# Autodesk Inventor assembly: Wheel Assembly
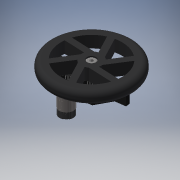
[picture p0: Inventor's stored thumbnail of the model, 180x180]
Saved by Autodesk Inventor 2017 (Build 210142000, 142)
## iProperties
Created: 2018-10-18
Part Number: Wheel Assembly
Document SubType Name: Assembly
Designer: Dell
Author: Dell
## Documents named in this file (7)
- C:\Users\Dell\Documents\GitHub\tr2\Wheel Assembly\Wheel Assembly.iam
- C:\Users\Dell\Documents\GitHub\tr2\Wheel Assembly\Scooter Wheel.ipt
- C:\Users\Dell\Documents\GitHub\tr2\Wheel Assembly\WA01.ipt
- C:\Users\Dell\Documents\GitHub\tr2\Wheel Assembly\Wheel Assembly\Design Accelerator\Spur Gears1.iam
- C:\Users\Dell\Documents\GitHub\tr2\Base\37d-gearmotor-50-70-encoder.ipt
- C:\Users\Dell\Documents\GitHub\tr2\Wheel Assembly\22x8x8mm Bearing.ipt
- C:\Users\Dell\Documents\GitHub\tr2\Wheel Assembly\6mm Mounting Hub, thin.ipt
## Components (10 placed, 6 different names)
1. Scooter Wheel:1 — Mate:8, Mate:25, Mate:26, Mate:27, Mate:28, Rotation:1
2. WA01:1 — Mate:9, Mate:10, Mate:11, Mate:24, Mate:31, Mate:33, Mate:35, Mate:36
3. Spur Gears:1 [sub-assembly] — Mate:8, Mate:17, Mate:19, Mate:21, Mate:22, Mate:31, Mate:32, Mate:33, Mate:38, Rotation:1
4. 37d-gearmotor-50-70-encoder:1 — Mate:9, Mate:10, Mate:11, Mate:20, Mate:32
5. 22x8x8mm Bearing:1 — Mate:17, Mate:37
6. 22x8x8mm Bearing:2 — Mate:19, Mate:36, Mate:37, Mate:38
7. 6mm Mounting Hub, thin:1 — Mate:20, Mate:21, Mate:22
8. 22x8x8mm Bearing:3 — Mate:24, Mate:34, Mate:35
9. 22x8x8mm Bearing:4 — Mate:25, Mate:26
10. 22x8x8mm Bearing:5 — Mate:27, Mate:28, Mate:34
## Relationships (23: Mate 22, RelateRotation 1)
- Mate:8: Scooter Wheel:1 ↔ Spur Gears:1
- Mate:9: WA01:1 ↔ 37d-gearmotor-50-70-encoder:1
- Mate:10: WA01:1 ↔ 37d-gearmotor-50-70-encoder:1
- Mate:11: WA01:1 ↔ 37d-gearmotor-50-70-encoder:1
- Mate:17: Spur Gears:1 ↔ 22x8x8mm Bearing:1
- Mate:19: Spur Gears:1 ↔ 22x8x8mm Bearing:2
- Mate:20: 37d-gearmotor-50-70-encoder:1 ↔ 6mm Mounting Hub, thin:1
- Mate:21: Spur Gears:1 ↔ 6mm Mounting Hub, thin:1
- Mate:22: Spur Gears:1 ↔ 6mm Mounting Hub, thin:1
- Mate:24: WA01:1 ↔ 22x8x8mm Bearing:3
- Mate:25: Scooter Wheel:1 ↔ 22x8x8mm Bearing:4
- Mate:26: Scooter Wheel:1 ↔ 22x8x8mm Bearing:4
- Mate:27: Scooter Wheel:1 ↔ 22x8x8mm Bearing:5
- Mate:28: Scooter Wheel:1 ↔ 22x8x8mm Bearing:5
- Mate:31: WA01:1 ↔ Spur Gears:1
- Mate:32: Spur Gears:1 ↔ 37d-gearmotor-50-70-encoder:1
- Mate:33: WA01:1 ↔ Spur Gears:1
- Mate:34: 22x8x8mm Bearing:3 ↔ 22x8x8mm Bearing:5
- Mate:35: WA01:1 ↔ 22x8x8mm Bearing:3
- Mate:36: WA01:1 ↔ 22x8x8mm Bearing:2
- Mate:37: 22x8x8mm Bearing:1 ↔ 22x8x8mm Bearing:2
- Mate:38: Spur Gears:1 ↔ 22x8x8mm Bearing:2
- Rotation:1 [RelateRotation] (1 ul): Scooter Wheel:1 ↔ Spur Gears:1
